# Autodesk Inventor assembly: Robot mrk3
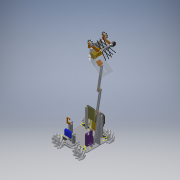
[picture p0: Inventor's stored thumbnail of the model, 180x180]
Saved by Autodesk Inventor 2019 (Build 230136000, 136)
## iProperties
Created: 2017-12-06
Part Number: Robot mrk3
Document SubType Name: Assembly
Designer: User
Author: User
## Documents named in this file (17)
- C:\Robotics\CAD\2018-19_CAD\Robot mrk2.iam
- C:\Robotics\CAD\2017-18_CAD\Prototypes\Gen2PlatePart.ipt
- C:\Robotics\CAD\2017-18_CAD\Prototypes\MecanumWheelFullForVexmotor.iam
- C:\Robotics\CAD\COTSParts\Rev\REV-41-1300HexMotor.ipt
- C:\Robotics\CAD\2017-18_CAD\Prototypes\MotorHolderA.ipt
- C:\Robotics\CAD\2017-18_CAD\Prototypes\MotorHolderB.ipt
- C:\Robotics\CAD\2018-19_CAD\Collection\20X20 lift.iam
- C:\Robotics\CAD\2018-19_CAD\Collection\SlidesPivotBracket.ipt
- C:\Robotics\CAD\2018-19_CAD\Collection\PaddleCollection2.1.ipt.iam
- C:\Robotics\CAD\2018-19_CAD\lift\lift assembly\Lead Screw Prototype A.iam
- C:\Robotics\CAD\2018-19_CAD\Collection\CollectionPost.ipt
- C:\Robotics\CAD\2018-19_CAD\Collection\paddle collection ramp.ipt
- C:\Robotics\CAD\2018-19_CAD\plate.iam
- C:\Robotics\CAD\2017-18_CAD\battery for holder.iam
- C:\Robotics\CAD\2018-19_CAD\3d printer\MotoGPhoneHolder.ipt
- C:\Robotics\CAD\COTSParts\Bosch Extrusion\Bosch 20x20 8.5inch.ipt
- PaddleCollection2.1.ipt
## Components (24 placed, 15 different names)
1. Gen2PlatePart:1 — Mate:12, Mate:14, Insert:9, Flush:30, Insert:13, Insert:14, Insert:21, Insert:22, Flush:34, Flush:36, Mate:34, Flush:37, Insert:27, Insert:28, Insert:29, Insert:30, Insert:31, Insert:32, Insert:33, Mate:36, Flush:41, Mate:37, Mate:38, Flush:42, Mate:41, Flush:43, Flush:45
2. MecanumWheelFullForVexmotor:1 [sub-assembly] — Insert:24, Rotation:2, Rotation:3
3. MecanumWheelFullForVexmotor:2 [sub-assembly] — Insert:11, Rotation:1
4. MecanumWheelFullForVexmotor:3 [sub-assembly] — Insert:23, Rotation:1, Rotation:3
5. REV-41-1300HexMotor:2 — Mate:12, Mate:24, Insert:23
6. REV-41-1300HexMotor:3 — Mate:14, Mate:20, Mate:21, Insert:24
7. REV-41-1300HexMotor:4 — Insert:11, Insert:20, Angle:1
8. MotorHolderA:1 — Mate:24, Insert:21, Insert:22
9. MotorHolderA:2 — Insert:9, Flush:30, Insert:25, Angle:2
10. MotorHolderB:1 — Mate:20, Mate:21
11. MotorHolderB:2 — Insert:13, Insert:14, Insert:20, Angle:1
12. REV-41-1300HexMotor:5 — Insert:25, Angle:2, Insert:26
13. MecanumWheelFullForVexmotor:4 [sub-assembly] — Insert:26, Rotation:2
14. SlidesPivotBracket:1 — Mate:31, Insert:27, Insert:28
15. SlidesPivotBracket:2 — Insert:29, Insert:30, Insert:31
16. 20X20 lift:2 [sub-assembly] — Mate:31, Flush:34, Mate:32, Mate:33, Flush:40
17. PaddleCollection2.1.ipt:1 [sub-assembly] — Mate:32, Mate:33, Flush:38, Mate:35, Flush:39, Flush:40
18. Lead Screw Prototype A:1 [sub-assembly] — Mate:34, Flush:37
19. CollectionPost:1 — Insert:32, Insert:33
20. paddle collection ramp:1 — Flush:38, Mate:35, Flush:39
21. plate:1 [sub-assembly] — Mate:36, Flush:41
22. battery for holder:1 [sub-assembly] — Mate:37, Mate:38, Flush:42
23. MotoGPhoneHolder:1 — Mate:42, Mate:43, Flush:43, Flush:44, Flush:45
24. Bosch 20x20 8.5inch:1 — Mate:41, Mate:42, Mate:43, Flush:44
## Relationships (51: Insert 18, Mate 16, Flush 12, RelateRotation 3, Angle 2)
- Mate:12: Gen2PlatePart:1 ↔ REV-41-1300HexMotor:2
- Mate:14: Gen2PlatePart:1 ↔ REV-41-1300HexMotor:3
- Mate:20: REV-41-1300HexMotor:3 ↔ MotorHolderB:1
- Mate:21: REV-41-1300HexMotor:3 ↔ MotorHolderB:1
- Mate:24: REV-41-1300HexMotor:2 ↔ MotorHolderA:1
- Insert:9: Gen2PlatePart:1 ↔ MotorHolderA:2
- Flush:30: Gen2PlatePart:1 ↔ MotorHolderA:2
- Insert:11: MecanumWheelFullForVexmotor:2 ↔ REV-41-1300HexMotor:4
- Insert:13: Gen2PlatePart:1 ↔ MotorHolderB:2
- Insert:14: Gen2PlatePart:1 ↔ MotorHolderB:2
- Insert:20: REV-41-1300HexMotor:4 ↔ MotorHolderB:2
- Angle:1 (180 deg): REV-41-1300HexMotor:4 ↔ MotorHolderB:2
- Insert:21: Gen2PlatePart:1 ↔ MotorHolderA:1
- Insert:22: Gen2PlatePart:1 ↔ MotorHolderA:1
- Insert:23: MecanumWheelFullForVexmotor:3 ↔ REV-41-1300HexMotor:2
- Insert:24: MecanumWheelFullForVexmotor:1 ↔ REV-41-1300HexMotor:3
- Insert:25: MotorHolderA:2 ↔ REV-41-1300HexMotor:5
- Angle:2 (0 deg): MotorHolderA:2 ↔ REV-41-1300HexMotor:5
- Insert:26: REV-41-1300HexMotor:5 ↔ MecanumWheelFullForVexmotor:4
- Rotation:1 [RelateRotation] (1 ul): MecanumWheelFullForVexmotor:2 ↔ MecanumWheelFullForVexmotor:3
- Rotation:2 [RelateRotation] (1 ul): MecanumWheelFullForVexmotor:1 ↔ MecanumWheelFullForVexmotor:4
- Rotation:3 [RelateRotation] (1 ul): MecanumWheelFullForVexmotor:1 ↔ MecanumWheelFullForVexmotor:3
- Mate:31: SlidesPivotBracket:1 ↔ 20X20 lift:2
- Flush:34 (117.0178 mm): Gen2PlatePart:1 ↔ 20X20 lift:2
- Mate:32: 20X20 lift:2 ↔ PaddleCollection2.1.ipt:1
- Mate:33: 20X20 lift:2 ↔ PaddleCollection2.1.ipt:1
- Flush:36 (360.0704 mm): Gen2PlatePart:1
- Mate:34: Gen2PlatePart:1 ↔ Lead Screw Prototype A:1
- Flush:37: Gen2PlatePart:1 ↔ Lead Screw Prototype A:1
- Insert:27: Gen2PlatePart:1 ↔ SlidesPivotBracket:1
- Insert:28: Gen2PlatePart:1 ↔ SlidesPivotBracket:1
- Insert:29: Gen2PlatePart:1 ↔ SlidesPivotBracket:2
- Insert:30: Gen2PlatePart:1 ↔ SlidesPivotBracket:2
- Insert:31: Gen2PlatePart:1 ↔ SlidesPivotBracket:2
- Insert:32: Gen2PlatePart:1 ↔ CollectionPost:1
- Insert:33: Gen2PlatePart:1 ↔ CollectionPost:1
- Flush:38: PaddleCollection2.1.ipt:1 ↔ paddle collection ramp:1
- Mate:35: PaddleCollection2.1.ipt:1 ↔ paddle collection ramp:1
- Flush:39 (1.27 mm): PaddleCollection2.1.ipt:1 ↔ paddle collection ramp:1
- Flush:40: 20X20 lift:2 ↔ PaddleCollection2.1.ipt:1
- Mate:36: Gen2PlatePart:1 ↔ plate:1
- Flush:41: Gen2PlatePart:1 ↔ plate:1
- Mate:37: Gen2PlatePart:1 ↔ battery for holder:1
- Mate:38: Gen2PlatePart:1 ↔ battery for holder:1
- Flush:42: Gen2PlatePart:1 ↔ battery for holder:1
- Mate:41: Gen2PlatePart:1 ↔ Bosch 20x20 8.5inch:1
- Mate:42: MotoGPhoneHolder:1 ↔ Bosch 20x20 8.5inch:1
- Mate:43 (3.048 mm): MotoGPhoneHolder:1 ↔ Bosch 20x20 8.5inch:1
- Flush:43: Gen2PlatePart:1 ↔ MotoGPhoneHolder:1
- Flush:44 (12.7 mm): MotoGPhoneHolder:1 ↔ Bosch 20x20 8.5inch:1
- Flush:45: Gen2PlatePart:1 ↔ MotoGPhoneHolder:1
